# Autodesk Inventor assembly: VMU on Camera Mount
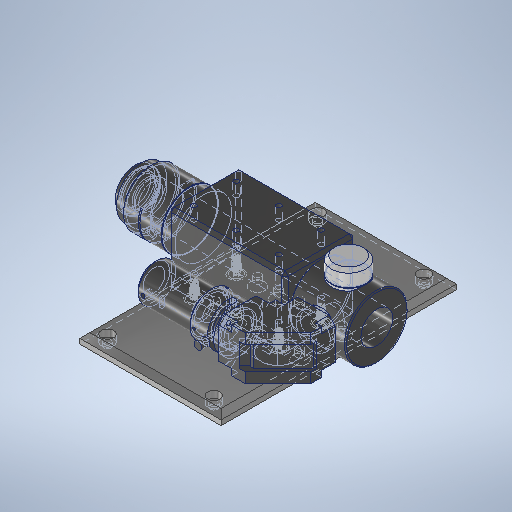
[picture p0: Inventor's stored thumbnail of the model, 512x512]
Saved by Autodesk Inventor 2025 (Build 290162000, 162)
## iProperties
Created: 2024-08-16
Part Number: VMU on Camera Mount
Document SubType Name: Assembly
Designer: Caleb Fangmeier
Author: Caleb Fangmeier
## Documents named in this file (4)
- C:\Users\cfang\Desktop\nebraska-silicon-lab\Hardware\General Gantry\Camera Mount\VMU on Camera Mount.iam
- C:\Users\cfang\Desktop\nebraska-silicon-lab\Hardware\General Gantry\Camera Mount\Mounting Plate.ipt
- C:\Users\cfang\Desktop\nebraska-silicon-lab\Hardware\General Gantry\Camera Mount\step_63024\step_63024.ipt
- C:\Users\cfang\Desktop\nebraska-silicon-lab\Hardware\General Gantry\Camera Mount\92010A220_Passivated 18-8 Stainless Steel Phillips Flat Head Screw\92010A220_Passivated 18-8 Stainless Steel Phillips Flat Head S.ipt
## Components (6 placed, 3 different names)
1. Mounting Plate:1 — Mate:1, Angle:1, Insert:1, Insert:2, Insert:3, Insert:4, Insert:5
2. step_63024:1 — Mate:1, Angle:1, Insert:1
3. 92010A220_Passivated 18-8 Stainless Steel Phillips Flat Head S:1 — Insert:4
4. 92010A220_Passivated 18-8 Stainless Steel Phillips Flat Head S:2 — Insert:5
5. 92010A220_Passivated 18-8 Stainless Steel Phillips Flat Head S:3 — Insert:2
6. 92010A220_Passivated 18-8 Stainless Steel Phillips Flat Head S:4 — Insert:3
## Relationships (7: Insert 5, Mate 1, Angle 1)
- Mate:1: Mounting Plate:1 ↔ step_63024:1
- Angle:1 (0 deg): Mounting Plate:1 ↔ step_63024:1
- Insert:1: Mounting Plate:1 ↔ step_63024:1
- Insert:2: Mounting Plate:1 ↔ 92010A220_Passivated 18-8 Stainless Steel Phillips Flat Head S:3
- Insert:3: Mounting Plate:1 ↔ 92010A220_Passivated 18-8 Stainless Steel Phillips Flat Head S:4
- Insert:4: Mounting Plate:1 ↔ 92010A220_Passivated 18-8 Stainless Steel Phillips Flat Head S:1
- Insert:5: Mounting Plate:1 ↔ 92010A220_Passivated 18-8 Stainless Steel Phillips Flat Head S:2
